# Autodesk Inventor assembly: 800-20-MOTOR-CONTROLLER-BLD-300B
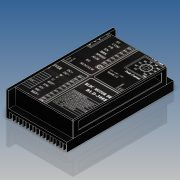
[picture p0: Inventor's stored thumbnail of the model, 180x180]
Saved by Autodesk Inventor 2018.2 (Build 222227000, 227)
## iProperties
Manager: feesmrt
Company: FRANCOR
Part Number: 800-20-MOTOR-CONTROLLER-BLD-300B
Project: Rescue Robot
Cost Center: -
Material: Generisch
Document SubType Name: Assembly
Designer: feesmrt
Engineer: feesmrt
Authority: feesmrt
Description: BLDC Motor Controller - BLD-300B
Stock Number: 800-20-MOTOR-CONTROLLER-BLD-300B
Subject: Rescue Robot
Author: feesmrt
Revision Number: 1
Title: BLDC Motor Controller - BLD-300B
## Documents named in this file (3)
- D:\Programmierung\FRANC0R\CAD\02-Rocker-Bogie-Robot\800-ELECTRONICS\800-20-MOTOR-CONTROLLER\800-20-MOTOR-CONTROLLER-BLD-300B.iam
- D:\Programmierung\FRANC0R\CAD\02-Rocker-Bogie-Robot\800-ELECTRONICS\800-20-MOTOR-CONTROLLER\800-20-MOTOR-CONTROLLER-BLD-300B-01.ipt
- D:\Programmierung\FRANC0R\CAD\02-Rocker-Bogie-Robot\800-ELECTRONICS\800-20-MOTOR-CONTROLLER\800-20-MOTOR-CONTROLLER-BLD-300B-02.ipt
## Components (2 placed, 2 different names)
1. 800-20-MOTOR-CONTROLLER-BLD-300B-01:1 — Passend:1, Passend:2, Fluchtend:1
2. 800-20-MOTOR-CONTROLLER-BLD-300B-02:1 — Passend:1, Passend:2, Fluchtend:1
## Relationships (3: Mate 2, Flush 1)
- Passend:1 [Mate]: 800-20-MOTOR-CONTROLLER-BLD-300B-01:1 ↔ 800-20-MOTOR-CONTROLLER-BLD-300B-02:1
- Passend:2 [Mate]: 800-20-MOTOR-CONTROLLER-BLD-300B-01:1 ↔ 800-20-MOTOR-CONTROLLER-BLD-300B-02:1
- Fluchtend:1 [Flush]: 800-20-MOTOR-CONTROLLER-BLD-300B-01:1 ↔ 800-20-MOTOR-CONTROLLER-BLD-300B-02:1
